# Autodesk Inventor assembly: Hing ass
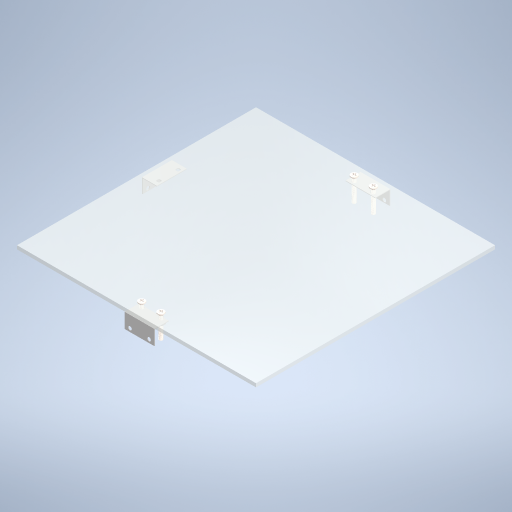
[picture p0: Inventor's stored thumbnail of the model, 512x512]
Saved by Autodesk Inventor 2024 (Build 280153000, 153)
## iProperties
Created: 2023-06-07
Part Number: Hing ass
Document SubType Name: Assembly
Designer: shrus
Author: shrus
## Documents named in this file (5)
- C:\Users\shraa\Downloads\Useless machine assembly\Hing ass.iam
- C:\Users\shraa\Downloads\Useless machine assembly\Hinge angle.ipt
- C:\Users\shraa\Downloads\Useless machine assembly\m3-6mm.ipt
- C:\Users\shraa\Downloads\Useless machine assembly\M3 Nut.ipt
- C:\Users\shraa\Downloads\Useless machine assembly\Topbottom.ipt
## Components (10 placed, 4 different names)
1. Topbottom:1 — Mate:1, Mate:2, Mate:5, Mate:6
2. Hinge angle:6 — Mate:3, Mate:4
3. m3-6mm:3 — Mate:2
4. m3-6mm:4 — Mate:1
5. M3 Nut:3 — Mate:4
6. M3 Nut:4 — Mate:3
7. Hinge angle:7
8. m3-6mm:5 — Mate:5
9. m3-6mm:6 — Mate:6
10. Hinge angle:9
## Relationships (6: Mate 6)
- Mate:1: Topbottom:1 ↔ m3-6mm:4
- Mate:2: Topbottom:1 ↔ m3-6mm:3
- Mate:3: Hinge angle:6 ↔ M3 Nut:4
- Mate:4: Hinge angle:6 ↔ M3 Nut:3
- Mate:5: Topbottom:1 ↔ m3-6mm:5
- Mate:6: Topbottom:1 ↔ m3-6mm:6
